# Autodesk Inventor assembly: tetrixDriver
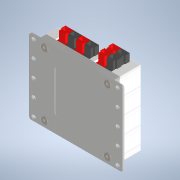
[picture p0: Inventor's stored thumbnail of the model, 180x180]
Saved by Autodesk Inventor 2022 (Build 260153000, 153)
## iProperties
Created: 2022-10-22
Part Number: tetrixDriver
Document SubType Name: Assembly
Designer: КозьминАндрей
Author: КозьминАндрей
## Documents named in this file (5)
- D:\Проэкты Autodesk Inventor\polivalka\tetrixDriver\tetrixDriver.iam
- D:\Проэкты Autodesk Inventor\polivalka\tetrixDriver\dno.ipt
- D:\Проэкты Autodesk Inventor\polivalka\tetrixDriver\krishka.ipt
- D:\Проэкты Autodesk Inventor\polivalka\tetrixDriver\vintik.ipt
- D:\Проэкты Autodesk Inventor\polivalka\tetrixDriver\vnutrennosti.ipt
## Components (7 placed, 4 different names)
1. dno:1 — Совмещение:1, Совмещение:2, Совмещение:3, Совмещение:4, Заподлицо:1, Заподлицо:2, Заподлицо:3, Совмещение:5, Заподлицо:4, Совмещение:6, Заподлицо:5, Совмещение:7, Заподлицо:6, Совмещение:8
2. krishka:1 — Совмещение:4, Заподлицо:1, Заподлицо:2
3. vnutrennosti:1 — Совмещение:1, Совмещение:2, Совмещение:3
4. vintik:1 — Заподлицо:6, Совмещение:8
5. vintik:2 — Заподлицо:3, Совмещение:5
6. vintik:3 — Заподлицо:4, Совмещение:6
7. vintik:4 — Заподлицо:5, Совмещение:7
## Relationships (14: Mate 8, Flush 6)
- Совмещение:1 [Mate]: dno:1 ↔ vnutrennosti:1
- Совмещение:2 [Mate]: dno:1 ↔ vnutrennosti:1
- Совмещение:3 [Mate]: dno:1 ↔ vnutrennosti:1
- Совмещение:4 [Mate]: dno:1 ↔ krishka:1
- Заподлицо:1 [Flush]: dno:1 ↔ krishka:1
- Заподлицо:2 [Flush]: dno:1 ↔ krishka:1
- Заподлицо:3 [Flush]: dno:1 ↔ vintik:2
- Совмещение:5 [Mate]: dno:1 ↔ vintik:2
- Заподлицо:4 [Flush]: dno:1 ↔ vintik:3
- Совмещение:6 [Mate]: dno:1 ↔ vintik:3
- Заподлицо:5 [Flush]: dno:1 ↔ vintik:4
- Совмещение:7 [Mate]: dno:1 ↔ vintik:4
- Заподлицо:6 [Flush]: dno:1 ↔ vintik:1
- Совмещение:8 [Mate]: dno:1 ↔ vintik:1
